# Autodesk Inventor assembly: moteur
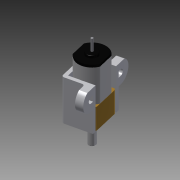
[picture p0: Inventor's stored thumbnail of the model, 180x180]
Saved by Autodesk Inventor 2014 SP2 (Build 180246200, 246)
## iProperties
Created: 2015-03-17
Part Number: moteur
Document SubType Name: Assembly
Designer: sd
Mass: 22.4502 g
Surface Area: 33.3553 cm^2
Volume: 3.85673 cm^3
Density: 5.82103 g/cm^3
Author: sd
## Documents named in this file (7)
- D:\Utilisateurs\sd\Mes documents\SVN\projets-gei\Dumber 2015\Mecanique\moteur.iam
- D:\Utilisateurs\sd\Mes documents\SVN\projets-gei\Dumber 2015\Mecanique\moteur.ipt
- D:\Utilisateurs\sd\Mes documents\SVN\projets-gei\Dumber 2015\Mecanique\axe.ipt
- D:\Utilisateurs\sd\Mes documents\SVN\projets-gei\Dumber 2015\Mecanique\plaque moteur.ipt
- D:\Utilisateurs\sd\Mes documents\SVN\projets-gei\Dumber 2015\Mecanique\queue.ipt
- D:\Utilisateurs\sd\Mes documents\SVN\projets-gei\Dumber 2015\Mecanique\reducteur.ipt
- D:\Utilisateurs\sd\Mes documents\SVN\projets-gei\Dumber 2015\Mecanique\fixation moteur.ipt
## Components (6 placed, 6 different names)
1. moteur:1 — Placage:1, Placage:2, Placage:3, Placage:6, Placage:7, Placage:8
2. axe:1 — Placage:4, Placage:5, Angle:1
3. plaque moteur:1 — Placage:6, Placage:7, Placage:8, Placage:9, Placage:10
4. queue:1 — Placage:9, Placage:10
5. reducteur:1 — Placage:1, Placage:2, Placage:3, Placage:4, Placage:5, Angle:1, Placage:11, Placage:12, Placage:13
6. fixation moteur:1 — Placage:11, Placage:12, Placage:13
## Relationships (14: Mate 13, Angle 1)
- Placage:1 [Mate]: moteur:1 ↔ reducteur:1
- Placage:2 [Mate]: moteur:1 ↔ reducteur:1
- Placage:3 [Mate]: moteur:1 ↔ reducteur:1
- Placage:4 [Mate]: axe:1 ↔ reducteur:1
- Placage:5 [Mate]: axe:1 ↔ reducteur:1
- Angle:1 (0 deg): axe:1 ↔ reducteur:1
- Placage:6 [Mate]: moteur:1 ↔ plaque moteur:1
- Placage:7 [Mate]: moteur:1 ↔ plaque moteur:1
- Placage:8 [Mate]: moteur:1 ↔ plaque moteur:1
- Placage:9 [Mate]: plaque moteur:1 ↔ queue:1
- Placage:10 [Mate]: plaque moteur:1 ↔ queue:1
- Placage:11 [Mate]: reducteur:1 ↔ fixation moteur:1
- Placage:12 [Mate]: reducteur:1 ↔ fixation moteur:1
- Placage:13 [Mate]: reducteur:1 ↔ fixation moteur:1
